# Autodesk Inventor assembly: HeadBasePt1
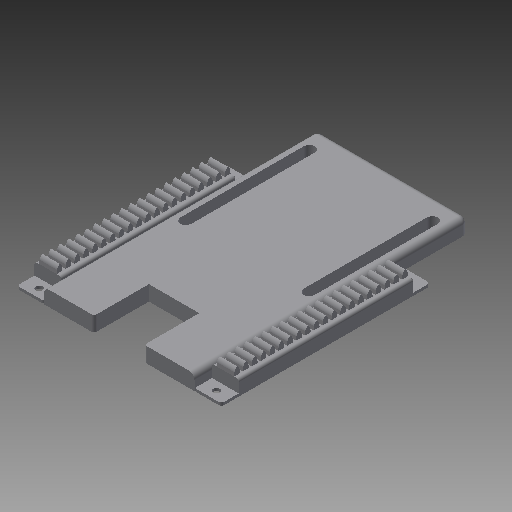
[picture p0: Inventor's stored thumbnail of the model, 512x512]
Saved by Autodesk Inventor 2018 (Build 220112000, 112)
## iProperties
Created: 2017-12-13
Part Number: HeadBasePt1
Document SubType Name: Assembly
Designer: reide
Author: reide
## Documents named in this file (3)
- C:\Users\reide\OneDrive\Documents\Inventor\TSA\2018\Animatronics\Tortoise\Head\HeadBasePt1.iam
- C:\Users\reide\OneDrive\Documents\Inventor\TSA\2018\Animatronics\Tortoise\Head\HeadBase.ipt
- C:\Users\reide\OneDrive\Documents\Inventor\TSA\2018\Animatronics\Tortoise\Rack.ipt
## Components (3 placed, 2 different names)
1. HeadBase:1 — Flush:1, Mate:1, Mate:2, Flush:4
2. Rack:1 — Flush:1, Mate:1
3. Rack:2 — Mate:2, Flush:4
## Relationships (4: Flush 2, Mate 2)
- Flush:1: HeadBase:1 ↔ Rack:1
- Mate:1: HeadBase:1 ↔ Rack:1
- Mate:2: HeadBase:1 ↔ Rack:2
- Flush:4: HeadBase:1 ↔ Rack:2
